# Autodesk Inventor assembly: Pump and motor Coupled
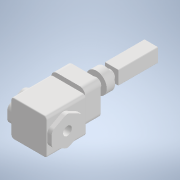
[picture p0: Inventor's stored thumbnail of the model, 180x180]
Saved by Autodesk Inventor 2020 (Build 240168000, 168)
## iProperties
Created: 2020-10-19
Part Number: Pump and motor Coupled
Document SubType Name: Assembly
Designer: jtri402
Author: jtri402
## Documents named in this file (4)
- \\files.auckland.ac.nz\myhome\Documents\CARMODEL\Pump and motor Coupled.iam
- \\files.auckland.ac.nz\myhome\Documents\CARMODEL\Electric Motor.ipt
- \\files.auckland.ac.nz\myhome\Documents\CARMODEL\Motor Pump.ipt
- \\files.auckland.ac.nz\myhome\Documents\CARMODEL\pump and e-motor coupling.ipt
## Components (3 placed, 3 different names)
1. Electric Motor:1 — Rigid:1
2. Motor Pump:1 — Rigid:2
3. pump and e-motor coupling:2 — Rigid:1, Rigid:2
## Relationships (2: WeldJoint 2)
- Rigid:1 [WeldJoint]: Electric Motor:1 ↔ pump and e-motor coupling:2
- Rigid:2 [WeldJoint]: Motor Pump:1 ↔ pump and e-motor coupling:2
